# Autodesk Inventor assembly: ASDSAssembly
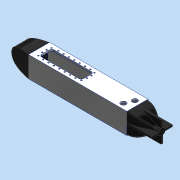
[picture p0: Inventor's stored thumbnail of the model, 180x180]
Saved by Autodesk Inventor 2018 (Build 220112000, 112)
## iProperties
Created: 2017-02-12
Part Number: ASDSAssembly
Document SubType Name: Assembly
Designer: techn
Author: techn
## Documents named in this file (4)
- D:\Projects\Submarine-project\CAD\ASDS\ASDSAssembly.iam
- D:\Projects\Submarine-project\CAD\ASDS\Fore.ipt
- D:\Projects\Submarine-project\CAD\ASDS\Aft.ipt
- D:\Projects\Submarine-project\CAD\ASDS\Hull_Alu.ipt
## Components (3 placed, 3 different names)
1. Fore:1 — Mate:1, Mate:2, Mate:3
2. Hull_Alu:1 — Mate:1, Mate:2, Mate:3, Mate:4, Mate:5, Mate:6
3. Aft:1 — Mate:4, Mate:5, Mate:6
## Relationships (6: Mate 6)
- Mate:1: Fore:1 ↔ Hull_Alu:1
- Mate:2: Fore:1 ↔ Hull_Alu:1
- Mate:3: Fore:1 ↔ Hull_Alu:1
- Mate:4: Hull_Alu:1 ↔ Aft:1
- Mate:5: Hull_Alu:1 ↔ Aft:1
- Mate:6: Hull_Alu:1 ↔ Aft:1
